# Autodesk Inventor assembly: rotor
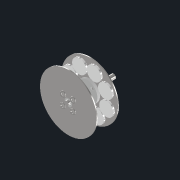
[picture p0: Inventor's stored thumbnail of the model, 180x180]
Saved by Autodesk Inventor 2022.2 (Build 262287010, 287A)
## iProperties
Created: 2023-07-19
Part Number: rotor
Document SubType Name: Assembly
Designer: StijnC
Author: StijnC
## Documents named in this file (6)
- C:\Users\techn\Desktop\AFM\V2\rotor.iam
- C:\Users\techn\Desktop\AFM\V2\magnet.ipt
- C:\Users\techn\Desktop\AFM\V2\plate.ipt
- C:\Users\techn\Desktop\AFM\V2\shaft.ipt
- C:\Users\techn\Desktop\AFM\V2\shaftmount.ipt
- C:\Users\techn\Documents\Inventor\Content Center Files\R2022\en-US\ANSI B18.3.4M(1)\ANSI B18.3.4M - M3 x 0.5 x 3(2).ipt
## Components (29 placed, 5 different names)
1. plate:1 — Mate:14, Mate:33, Mate:36, Mate:40, Insert:1, Insert:2, Insert:3, Insert:4
2. shaft:1 — Mate:14, Mate:15, Mate:31, Mate:32, Mate:41, Flush:4
3. plate:2 — Mate:15, Mate:18, Mate:19, Mate:34, Mate:37, Insert:5, Insert:6, Insert:7, Insert:8
4. shaftmount:1 — Mate:32, Mate:34, Mate:35, Mate:37, Angle:9
5. shaftmount:2 — Mate:31, Mate:33, Mate:35, Mate:36, Flush:4, Angle:7
6. Broached Hexagon Socket Button Head Cap Screw - Metric M3 x 0.5 x 3:1 — Insert:3, Angle:5, Angle:6
7. Broached Hexagon Socket Button Head Cap Screw - Metric M3 x 0.5 x 3:2 — Insert:1, Angle:6, Angle:7
8. Broached Hexagon Socket Button Head Cap Screw - Metric M3 x 0.5 x 3:3 — Insert:2, Angle:4
9. Broached Hexagon Socket Button Head Cap Screw - Metric M3 x 0.5 x 3:4 — Insert:4, Angle:4, Angle:5
10. Broached Hexagon Socket Button Head Cap Screw - Metric M3 x 0.5 x 3:5 — Insert:6, Angle:2, Angle:3
11. Broached Hexagon Socket Button Head Cap Screw - Metric M3 x 0.5 x 3:6 — Insert:5, Angle:2
12. Broached Hexagon Socket Button Head Cap Screw - Metric M3 x 0.5 x 3:7 — Insert:7, Angle:3, Angle:8, Angle:9
13. Broached Hexagon Socket Button Head Cap Screw - Metric M3 x 0.5 x 3:8 — Insert:8, Angle:8
14. magnet:2 — Mate:18, Mate:19
15. magnet:3
16. magnet:4
17. magnet:5
18. magnet:6
19. magnet:7
20. magnet:8 — Mate:42
21. magnet:9
22. magnet:10 — Mate:40, Mate:41, Mate:42
23. magnet:11
24. magnet:12
25. magnet:13
26. magnet:14
27. magnet:15
28. magnet:16
29. magnet:17
## Component patterns: (8 elements, first: magnet:2), (8 elements, first: magnet:10)
## Relationships (31: Mate 14, Insert 8, Angle 8, Flush 1)
- Mate:14: plate:1 ↔ shaft:1
- Mate:15: shaft:1 ↔ plate:2
- Mate:18: plate:2 ↔ magnet:2
- Mate:19 (20.5 mm): plate:2 ↔ magnet:2
- Mate:31: shaft:1 ↔ shaftmount:2
- Mate:32: shaft:1 ↔ shaftmount:1
- Mate:33: plate:1 ↔ shaftmount:2
- Mate:34: plate:2 ↔ shaftmount:1
- Mate:35: shaftmount:1 ↔ shaftmount:2
- Mate:36: plate:1 ↔ shaftmount:2
- Mate:37: plate:2 ↔ shaftmount:1
- Mate:40: plate:1 ↔ magnet:10
- Mate:41 (20.5 mm): shaft:1 ↔ magnet:10
- Mate:42: magnet:8 ↔ magnet:10
- Flush:4 (-2 mm): shaft:1 ↔ shaftmount:2
- Insert:1: plate:1 ↔ Broached Hexagon Socket Button Head Cap Screw - Metric M3 x 0.5 x 3:2
- Insert:2: plate:1 ↔ Broached Hexagon Socket Button Head Cap Screw - Metric M3 x 0.5 x 3:3
- Insert:3: plate:1 ↔ Broached Hexagon Socket Button Head Cap Screw - Metric M3 x 0.5 x 3:1
- Insert:4: plate:1 ↔ Broached Hexagon Socket Button Head Cap Screw - Metric M3 x 0.5 x 3:4
- Insert:5: plate:2 ↔ Broached Hexagon Socket Button Head Cap Screw - Metric M3 x 0.5 x 3:6
- Insert:6: plate:2 ↔ Broached Hexagon Socket Button Head Cap Screw - Metric M3 x 0.5 x 3:5
- Insert:7: plate:2 ↔ Broached Hexagon Socket Button Head Cap Screw - Metric M3 x 0.5 x 3:7
- Insert:8: plate:2 ↔ Broached Hexagon Socket Button Head Cap Screw - Metric M3 x 0.5 x 3:8
- Angle:2 (0 deg): Broached Hexagon Socket Button Head Cap Screw - Metric M3 x 0.5 x 3:5 ↔ Broached Hexagon Socket Button Head Cap Screw - Metric M3 x 0.5 x 3:6
- Angle:3 (0 deg): Broached Hexagon Socket Button Head Cap Screw - Metric M3 x 0.5 x 3:5 ↔ Broached Hexagon Socket Button Head Cap Screw - Metric M3 x 0.5 x 3:7
- Angle:4 (0 deg): Broached Hexagon Socket Button Head Cap Screw - Metric M3 x 0.5 x 3:3 ↔ Broached Hexagon Socket Button Head Cap Screw - Metric M3 x 0.5 x 3:4
- Angle:5 (0 deg): Broached Hexagon Socket Button Head Cap Screw - Metric M3 x 0.5 x 3:1 ↔ Broached Hexagon Socket Button Head Cap Screw - Metric M3 x 0.5 x 3:4
- Angle:6 (0 deg): Broached Hexagon Socket Button Head Cap Screw - Metric M3 x 0.5 x 3:1 ↔ Broached Hexagon Socket Button Head Cap Screw - Metric M3 x 0.5 x 3:2
- Angle:7 (0 deg): shaftmount:2 ↔ Broached Hexagon Socket Button Head Cap Screw - Metric M3 x 0.5 x 3:2
- Angle:8 (0 deg): Broached Hexagon Socket Button Head Cap Screw - Metric M3 x 0.5 x 3:7 ↔ Broached Hexagon Socket Button Head Cap Screw - Metric M3 x 0.5 x 3:8
- Angle:9 (0 deg): shaftmount:1 ↔ Broached Hexagon Socket Button Head Cap Screw - Metric M3 x 0.5 x 3:7
